# Autodesk Inventor assembly: main_assembly
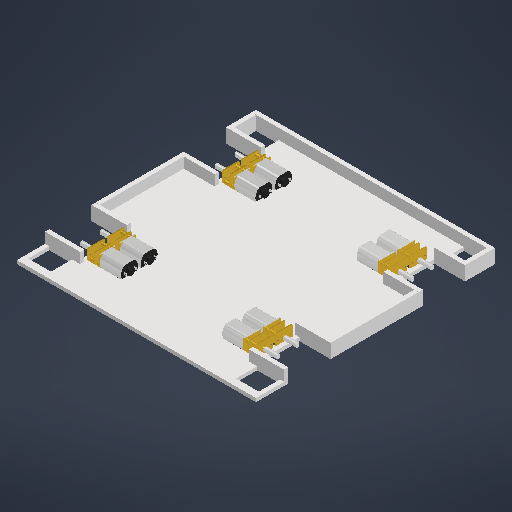
[picture p0: Inventor's stored thumbnail of the model, 512x512]
Saved by Autodesk Inventor 2026.2 (Build 302298010, 298A)
## iProperties
Created: 2026-03-12
Part Number: main_assembly
Document SubType Name: Assembly
Designer: karol
Author: karol
## Documents named in this file (11)
- C:\Users\karol\OneDrive\Desktop\robo\bolt\cad\assembly\main_assembly.iam
- C:\Users\karol\OneDrive\Desktop\robo\bolt\cad\assembly\base+motors.iam
- C:\Users\karol\OneDrive\Desktop\robo\bolt\cad\ready parts\backwall.ipt
- C:\Users\karol\OneDrive\Desktop\robo\bolt\cad\ready parts\left\left backside.ipt
- C:\Users\karol\OneDrive\Desktop\robo\bolt\cad\ready parts\right\right backside.ipt
- C:\Users\karol\OneDrive\Desktop\robo\bolt\cad\ready parts\right\roght backbackmotorwall.ipt
- C:\Users\karol\OneDrive\Desktop\robo\bolt\cad\ready parts\left\left backbackmotorwall.ipt
- C:\Users\karol\OneDrive\Desktop\robo\bolt\cad\ready parts\left\left back front motorwall; front, back and front motrowall.ipt
- C:\Users\karol\OneDrive\Desktop\robo\bolt\cad\ready parts\left\left sidewall.ipt
- C:\Users\karol\OneDrive\Desktop\robo\bolt\cad\ready parts\right\right back front motorwall; front, back and front motrowall.ipt
- C:\Users\karol\OneDrive\Desktop\robo\bolt\cad\ready parts\right\right sidewall.ipt
## Components (14 placed, 10 different names)
1. base+motors:1 [sub-assembly] — Mate:1, Mate:2, Mate:3, Mate:4, Mate:5, Mate:6, Mate:7, Mate:9, Mate:11, Mate:12, Mate:13, Mate:14, Mate:15, Mate:16, Mate:17, Mate:19, Mate:20, Mate:21, Mate:22, Mate:23, Mate:24, Mate:25
2. backwall:1 — Mate:1, Mate:2
3. left backside:1 — Mate:3, Mate:4, Mate:10
4. right backside:1 — Mate:5, Mate:6, Mate:8
5. roght backbackmotorwall:1 — Mate:7, Mate:8
6. left backbackmotorwall:1 — Mate:9, Mate:10
7. left back front motorwall; front, back and front motrowall:1 — Mate:11, Mate:12
8. left back front motorwall; front, back and front motrowall:2 — Mate:15, Mate:16
9. left back front motorwall; front, back and front motrowall:3 — Mate:13, Mate:14, Mate:18
10. left sidewall:1 — Mate:17, Mate:18
11. right back front motorwall; front, back and front motrowall:1 — Mate:19, Mate:20, Mate:26
12. right back front motorwall; front, back and front motrowall:2 — Mate:21, Mate:22
13. right back front motorwall; front, back and front motrowall:3 — Mate:23, Mate:24
14. right sidewall:1 — Mate:25, Mate:26
## Relationships (26: Mate 26)
- Mate:1: base+motors:1 ↔ backwall:1
- Mate:2: base+motors:1 ↔ backwall:1
- Mate:3: base+motors:1 ↔ left backside:1
- Mate:4: base+motors:1 ↔ left backside:1
- Mate:5: base+motors:1 ↔ right backside:1
- Mate:6: base+motors:1 ↔ right backside:1
- Mate:7: base+motors:1 ↔ roght backbackmotorwall:1
- Mate:8: right backside:1 ↔ roght backbackmotorwall:1
- Mate:9: base+motors:1 ↔ left backbackmotorwall:1
- Mate:10: left backside:1 ↔ left backbackmotorwall:1
- Mate:11: base+motors:1 ↔ left back front motorwall; front, back and front motrowall:1
- Mate:12: base+motors:1 ↔ left back front motorwall; front, back and front motrowall:1
- Mate:13: base+motors:1 ↔ left back front motorwall; front, back and front motrowall:3
- Mate:14: base+motors:1 ↔ left back front motorwall; front, back and front motrowall:3
- Mate:15: base+motors:1 ↔ left back front motorwall; front, back and front motrowall:2
- Mate:16: base+motors:1 ↔ left back front motorwall; front, back and front motrowall:2
- Mate:17: base+motors:1 ↔ left sidewall:1
- Mate:18: left back front motorwall; front, back and front motrowall:3 ↔ left sidewall:1
- Mate:19: base+motors:1 ↔ right back front motorwall; front, back and front motrowall:1
- Mate:20: base+motors:1 ↔ right back front motorwall; front, back and front motrowall:1
- Mate:21: base+motors:1 ↔ right back front motorwall; front, back and front motrowall:2
- Mate:22: base+motors:1 ↔ right back front motorwall; front, back and front motrowall:2
- Mate:23: base+motors:1 ↔ right back front motorwall; front, back and front motrowall:3
- Mate:24: base+motors:1 ↔ right back front motorwall; front, back and front motrowall:3
- Mate:25: base+motors:1 ↔ right sidewall:1
- Mate:26: right back front motorwall; front, back and front motrowall:1 ↔ right sidewall:1
